# Autodesk Inventor assembly: Ch-0-02-ChassisFrame
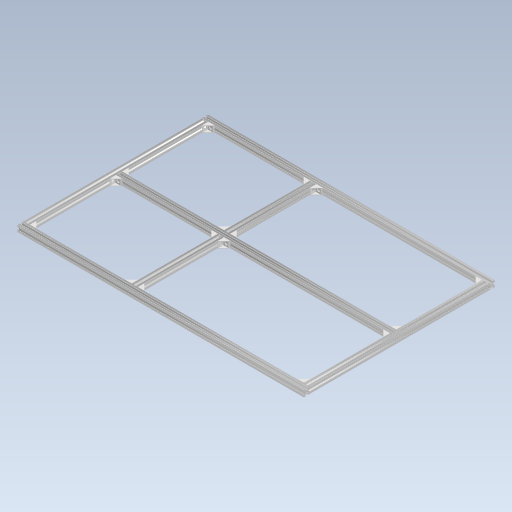
[picture p0: Inventor's stored thumbnail of the model, 512x512]
Saved by Autodesk Inventor 2023 (Build 270158000, 158)
## iProperties
Created: 2023-02-17
Part Number: Ch-0-02-ChassisFrame
Document SubType Name: Assembly
Designer: Dave
Author: Dave
## Documents named in this file (10)
- C:\Users\Dave\Documents\GitHub\BehrendURCMechanical\CAD\Chassis\Ch-0-02-ChassisFrame.iam
- C:\Users\Dave\Documents\GitHub\BehrendURCMechanical\CAD\Chassis\CH-1-01-20x20 Channel\CH-1-01-20x20 Channel-900.ipt
- C:\Users\Dave\Documents\GitHub\BehrendURCMechanical\CAD\Chassis\CH-1-01-20x20 Channel.ipt
- C:\Users\Dave\Documents\GitHub\BehrendURCMechanical\CAD\Chassis\CH-1-01-20x20 Channel\20x20 Channel-560.ipt
- C:\Users\Dave\Documents\GitHub\BehrendURCMechanical\CAD\Chassis\CH-1-01-20x20 Channel\CH-1-01-20x20 Channel-860.ipt
- C:\Users\Dave\Documents\GitHub\BehrendURCMechanical\CAD\Chassis\CH-1-01-20x20 Channel\CH-1-01-20x20 Channel-270.ipt
- C:\Users\Dave\Documents\GitHub\BehrendURCMechanical\CAD\Chassis\CH-1-01-Cornerbracket.ipt
- C:\Users\Dave\Documents\GitHub\BehrendURCMechanical\CAD\Chassis\CH-1-01-Cornerbracket1.ipt
- C:\Users\Dave\Documents\GitHub\BehrendURCMechanical\CAD\Chassis\CH-1-01-Cornerbracket2.ipt
- C:\Users\Dave\Documents\GitHub\BehrendURCMechanical\CAD\Chassis\CH-1-01-Cornerbracket11.ipt
## Components (23 placed, 8 different names)
1. CH-1-01-20x20 Channel-900:1 — Flush:4, Flush:6, Mate:5, Flush:8, Mate:8, Mate:10, Flush:25, Flush:26, Flush:27, Mate:36, Mate:37, Mate:40, Mate:41
2. CH-1-01-20x20 Channel-900:2 — Flush:3, Flush:5, Mate:7, Flush:9, Flush:10, Mate:9, Flush:11, Flush:12, Flush:13, Flush:14, Mate:12, Mate:13, Mate:15, Mate:18, Flush:15
3. 20x20 Channel-560:5 — Mate:3, Flush:2, Flush:3, Flush:4, Flush:8, Flush:9, Mate:10, Mate:11, Mate:19, Mate:22, Mate:42
4. 20x20 Channel-560:6 — Flush:5, Mate:4, Flush:10, Mate:8, Mate:9, Mate:17, Flush:28, Mate:32, Mate:34, Mate:35
5. CH-1-01-20x20 Channel-860:7 — Mate:1, Mate:2, Flush:1, Mate:3, Flush:2, Mate:4, Mate:6, Flush:7, Flush:16, Flush:17, Flush:22, Flush:23, Mate:20, Mate:21, Mate:24, Mate:26, Mate:27, Mate:30, Mate:31, Mate:33
6. CH-1-01-20x20 Channel-270:8 — Flush:6, Mate:5, Mate:28, Mate:29, Mate:38, Mate:39, Flush:29
7. CH-1-01-20x20 Channel-270:9 — Mate:6, Flush:7, Mate:7, Mate:14, Mate:16, Mate:23, Mate:25, Flush:29
8. CH-1-01-Cornerbracket:1 — Flush:14, Mate:11, Mate:12
9. CH-1-01-Cornerbracket:2 — Flush:11, Mate:13, Mate:14
10. CH-1-01-Cornerbracket:3 — Flush:12, Mate:15, Mate:16
11. CH-1-01-Cornerbracket:4 — Flush:13, Mate:17, Mate:18
12. CH-1-01-Cornerbracket1:1 — Flush:16, Mate:19, Mate:20
13. CH-1-01-Cornerbracket1:2 — Flush:18, Flush:23, Mate:23, Mate:24
14. CH-1-01-Cornerbracket1:3 — Flush:20, Mate:25, Mate:26
15. CH-1-01-Cornerbracket1:4 — Flush:21, Flush:22, Mate:33, Mate:34
16. CH-1-01-Cornerbracket2:1 — Flush:25, Mate:41, Mate:42
17. CH-1-01-Cornerbracket2:2 — Flush:26, Mate:39, Mate:40
18. CH-1-01-Cornerbracket2:3 — Flush:27, Mate:37, Mate:38
19. CH-1-01-Cornerbracket2:4 — Flush:28, Mate:35, Mate:36
20. CH-1-01-Cornerbracket11:1 — Flush:17, Mate:21, Mate:22
21. CH-1-01-Cornerbracket11:2 — Flush:18, Flush:19, Mate:27, Mate:28
22. CH-1-01-Cornerbracket11:3 — Flush:19, Flush:20, Mate:29, Mate:30
23. CH-1-01-Cornerbracket11:4 — Flush:21, Mate:31, Mate:32
## Relationships (70: Mate 42, Flush 28)
- Mate:1: CH-1-01-20x20 Channel-860:7
- Mate:2 (-10 mm): CH-1-01-20x20 Channel-860:7
- Flush:1: CH-1-01-20x20 Channel-860:7
- Mate:3: 20x20 Channel-560:5 ↔ CH-1-01-20x20 Channel-860:7
- Flush:2: 20x20 Channel-560:5 ↔ CH-1-01-20x20 Channel-860:7
- Flush:3: CH-1-01-20x20 Channel-900:2 ↔ 20x20 Channel-560:5
- Flush:4: CH-1-01-20x20 Channel-900:1 ↔ 20x20 Channel-560:5
- Flush:5: CH-1-01-20x20 Channel-900:2 ↔ 20x20 Channel-560:6
- Mate:4: 20x20 Channel-560:6 ↔ CH-1-01-20x20 Channel-860:7
- Flush:6: CH-1-01-20x20 Channel-900:1 ↔ CH-1-01-20x20 Channel-270:8
- Mate:5: CH-1-01-20x20 Channel-900:1 ↔ CH-1-01-20x20 Channel-270:8
- Mate:6: CH-1-01-20x20 Channel-860:7 ↔ CH-1-01-20x20 Channel-270:9
- Flush:7: CH-1-01-20x20 Channel-860:7 ↔ CH-1-01-20x20 Channel-270:9
- Mate:7: CH-1-01-20x20 Channel-900:2 ↔ CH-1-01-20x20 Channel-270:9
- Flush:8: CH-1-01-20x20 Channel-900:1 ↔ 20x20 Channel-560:5
- Flush:9: CH-1-01-20x20 Channel-900:2 ↔ 20x20 Channel-560:5
- Flush:10: CH-1-01-20x20 Channel-900:2 ↔ 20x20 Channel-560:6
- Mate:8: CH-1-01-20x20 Channel-900:1 ↔ 20x20 Channel-560:6
- Mate:9: CH-1-01-20x20 Channel-900:2 ↔ 20x20 Channel-560:6
- Mate:10: CH-1-01-20x20 Channel-900:1 ↔ 20x20 Channel-560:5
- Flush:11: CH-1-01-20x20 Channel-900:2 ↔ CH-1-01-Cornerbracket:2
- Flush:12: CH-1-01-20x20 Channel-900:2 ↔ CH-1-01-Cornerbracket:3
- Flush:13: CH-1-01-20x20 Channel-900:2 ↔ CH-1-01-Cornerbracket:4
- Flush:14: CH-1-01-20x20 Channel-900:2 ↔ CH-1-01-Cornerbracket:1
- Mate:11: 20x20 Channel-560:5 ↔ CH-1-01-Cornerbracket:1
- Mate:12: CH-1-01-20x20 Channel-900:2 ↔ CH-1-01-Cornerbracket:1
- Mate:13: CH-1-01-20x20 Channel-900:2 ↔ CH-1-01-Cornerbracket:2
- Mate:14: CH-1-01-20x20 Channel-270:9 ↔ CH-1-01-Cornerbracket:2
- Mate:15: CH-1-01-20x20 Channel-900:2 ↔ CH-1-01-Cornerbracket:3
- Mate:16: CH-1-01-20x20 Channel-270:9 ↔ CH-1-01-Cornerbracket:3
- Mate:17: 20x20 Channel-560:6 ↔ CH-1-01-Cornerbracket:4
- Mate:18: CH-1-01-20x20 Channel-900:2 ↔ CH-1-01-Cornerbracket:4
- Flush:15 (135 mm): CH-1-01-20x20 Channel-900:2
- Flush:16: CH-1-01-20x20 Channel-860:7 ↔ CH-1-01-Cornerbracket1:1
- Flush:17: CH-1-01-20x20 Channel-860:7 ↔ CH-1-01-Cornerbracket11:1
- Flush:18: CH-1-01-Cornerbracket1:2 ↔ CH-1-01-Cornerbracket11:2
- Flush:19: CH-1-01-Cornerbracket11:2 ↔ CH-1-01-Cornerbracket11:3
- Flush:20: CH-1-01-Cornerbracket1:3 ↔ CH-1-01-Cornerbracket11:3
- Flush:21: CH-1-01-Cornerbracket1:4 ↔ CH-1-01-Cornerbracket11:4
- Flush:22: CH-1-01-20x20 Channel-860:7 ↔ CH-1-01-Cornerbracket1:4
- Flush:23: CH-1-01-20x20 Channel-860:7 ↔ CH-1-01-Cornerbracket1:2
- Flush:25: CH-1-01-20x20 Channel-900:1 ↔ CH-1-01-Cornerbracket2:1
- Flush:26: CH-1-01-20x20 Channel-900:1 ↔ CH-1-01-Cornerbracket2:2
- Flush:27: CH-1-01-20x20 Channel-900:1 ↔ CH-1-01-Cornerbracket2:3
- Flush:28: 20x20 Channel-560:6 ↔ CH-1-01-Cornerbracket2:4
- Mate:19: 20x20 Channel-560:5 ↔ CH-1-01-Cornerbracket1:1
- Mate:20: CH-1-01-20x20 Channel-860:7 ↔ CH-1-01-Cornerbracket1:1
- Mate:21: CH-1-01-20x20 Channel-860:7 ↔ CH-1-01-Cornerbracket11:1
- Mate:22: 20x20 Channel-560:5 ↔ CH-1-01-Cornerbracket11:1
- Mate:23: CH-1-01-20x20 Channel-270:9 ↔ CH-1-01-Cornerbracket1:2
- Mate:24: CH-1-01-20x20 Channel-860:7 ↔ CH-1-01-Cornerbracket1:2
- Mate:25: CH-1-01-20x20 Channel-270:9 ↔ CH-1-01-Cornerbracket1:3
- Mate:26: CH-1-01-20x20 Channel-860:7 ↔ CH-1-01-Cornerbracket1:3
- Mate:27: CH-1-01-20x20 Channel-860:7 ↔ CH-1-01-Cornerbracket11:2
- Mate:28: CH-1-01-20x20 Channel-270:8 ↔ CH-1-01-Cornerbracket11:2
- Mate:29: CH-1-01-20x20 Channel-270:8 ↔ CH-1-01-Cornerbracket11:3
- Mate:30: CH-1-01-20x20 Channel-860:7 ↔ CH-1-01-Cornerbracket11:3
- Mate:31: CH-1-01-20x20 Channel-860:7 ↔ CH-1-01-Cornerbracket11:4
- Mate:32: 20x20 Channel-560:6 ↔ CH-1-01-Cornerbracket11:4
- Mate:33: CH-1-01-20x20 Channel-860:7 ↔ CH-1-01-Cornerbracket1:4
- Mate:34: 20x20 Channel-560:6 ↔ CH-1-01-Cornerbracket1:4
- Mate:35: 20x20 Channel-560:6 ↔ CH-1-01-Cornerbracket2:4
- Mate:36: CH-1-01-20x20 Channel-900:1 ↔ CH-1-01-Cornerbracket2:4
- Mate:37: CH-1-01-20x20 Channel-900:1 ↔ CH-1-01-Cornerbracket2:3
- Mate:38: CH-1-01-20x20 Channel-270:8 ↔ CH-1-01-Cornerbracket2:3
- Mate:39: CH-1-01-20x20 Channel-270:8 ↔ CH-1-01-Cornerbracket2:2
- Mate:40: CH-1-01-20x20 Channel-900:1 ↔ CH-1-01-Cornerbracket2:2
- Mate:41: CH-1-01-20x20 Channel-900:1 ↔ CH-1-01-Cornerbracket2:1
- Mate:42: 20x20 Channel-560:5 ↔ CH-1-01-Cornerbracket2:1
- Flush:29: CH-1-01-20x20 Channel-270:8 ↔ CH-1-01-20x20 Channel-270:9
